# Autodesk Inventor assembly: ASY ДМФ лоток 050 илоотвод
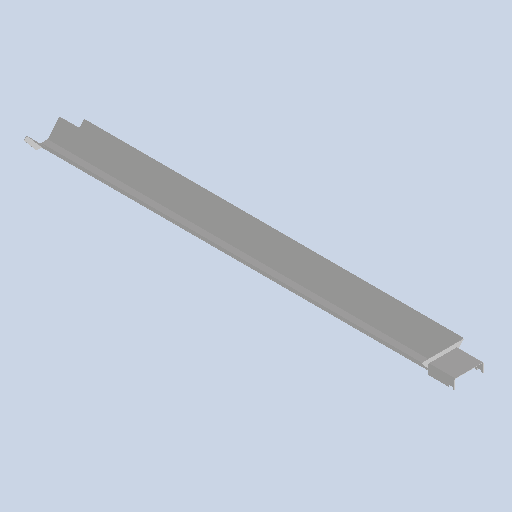
[picture p0: Inventor's stored thumbnail of the model, 512x512]
Saved by Autodesk Inventor 2025 (Build 290162010, 162A)
## iProperties
Created: 2024-05-14
Part Number: ASY ДМФ лоток 050 илоотвод
Document SubType Name: Assembly
Designer: admin
Author: admin
## Documents named in this file (5)
- C:\Users\pokla\Documents\Inventor\ДФО\ДМФ\DMF-Disk-Micro-Filter\DMF old version\ASY ДМФ лоток 050 илоотвод.iam
- C:\Users\pokla\Documents\Inventor\ДФО\ДМФ\DMF-Disk-Micro-Filter\DMF old version\ДМФ 051 лоток илоотвод.ipt
- C:\Users\pokla\Documents\Inventor\ДФО\ДМФ\DMF-Disk-Micro-Filter\DMF old version\ДМФ 052 торец лотка кормовой.ipt
- C:\Users\pokla\Documents\Inventor\ДФО\ДМФ\DMF-Disk-Micro-Filter\DMF old version\ДМФ 053 швеллер лотка.ipt
- C:\Users\pokla\Documents\Inventor\ДФО\ДМФ\DMF-Disk-Micro-Filter\DMF old version\ДМФ 054 фланец лотка.ipt
## Components (4 placed, 4 different names)
1. ДМФ 051 лоток илоотвод.ipt:1
2. ДМФ 052 торец лотка кормовой.ipt:1 — Flush:1, Mate:1
3. ДМФ 053 швеллер лотка.ipt:1 — Flush:1, Mate:1, Flush:2
4. ДМФ 054 фланец лотка.ipt:1
## Relationships (5: WeldJoint 2, Flush 2, Mate 1)
- [WeldJoint]: ДМФ 051 лоток илоотвод.ipt:1 ↔ ДМФ 052 торец лотка кормовой.ipt:1
- [WeldJoint]: ДМФ 051 лоток илоотвод.ipt:1 ↔ ДМФ 054 фланец лотка.ipt:1
- Flush:1 (20 mm): ДМФ 052 торец лотка кормовой.ipt:1 ↔ ДМФ 053 швеллер лотка.ipt:1
- Mate:1: ДМФ 052 торец лотка кормовой.ipt:1 ↔ ДМФ 053 швеллер лотка.ipt:1
- Flush:2: ДМФ 053 швеллер лотка.ipt:1
